# Autodesk Inventor assembly: use this - gimme that tech award
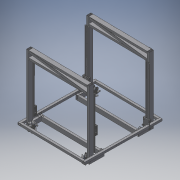
[picture p0: Inventor's stored thumbnail of the model, 180x180]
Saved by Autodesk Inventor 2018 (Build 220112000, 112)
## iProperties
Created: 2019-01-10
Part Number: use this - gimme that tech award
Document SubType Name: Assembly
Designer: maste
Author: maste
## Documents named in this file (7)
- \\studenthome\students\S-2512711\GitHub\2019CAD\Drivebase but Calvin is a mad man\use this - gimme that tech award.iam
- \\studenthome\students\S-2512711\GitHub\2019CAD\Drivebase but Calvin is a mad man\Slidey Mecanum L thing V2.iam
- \\studenthome\students\S-2512711\GitHub\2019CAD\Drivebase but Calvin is a mad man\1x1 30in.ipt
- \\studenthome\students\S-2512711\GitHub\2019CAD\Drivebase but Calvin is a mad man\1x1 35in.ipt
- \\studenthome\students\S-2512711\GitHub\2019CAD\Drivebase but Calvin is a mad man\1x1 L brackets 2in.ipt
- \\studenthome\students\S-2512711\GitHub\2019CAD\Drivebase but Calvin is a mad man\98404A101_18-8 STAINLESS STEEL QUICK-RELEASE PIN.ipt
- \\studenthome\students\S-2512711\GitHub\2019CAD\Drivebase but Calvin is a mad man\WW_10_40_10_AL_2.ipt
## Components (18 placed, 6 different names)
1. Slidey Mecanum L thing V2:1 [sub-assembly] — Mate:29, Mate:30, Flush:20, Flush:22, Flush:24, Mate:54, Mate:59, Mate:60, Mate:61, Mate:62
2. Slidey Mecanum L thing V2:2 [sub-assembly] — Flush:21, Mate:42, Flush:23, Mate:53, Flush:29, Mate:55, Mate:56, Mate:57, Mate:58
3. 1x1 30in:1 — Mate:31, Mate:32, Mate:33, Mate:34, Mate:35, Mate:36
4. 1x1 30in:2 — Mate:37, Mate:38, Mate:39, Flush:29
5. 1x1 35in:1 — Mate:29, Mate:30, Flush:20, Mate:31, Mate:32, Mate:33, Mate:45, Mate:46, Mate:47, Mate:48, Mate:54
6. 1x1 35in:2 — Mate:34, Mate:35, Mate:36, Mate:37, Mate:38, Mate:39, Mate:40, Mate:41, Mate:42, Mate:43, Mate:44, Mate:53
7. 1x1 L brackets 2in:1 — Flush:22, Mate:43, Mate:44, Mate:50, Flush:27, Rotation:2
8. 1x1 L brackets 2in:2 — Mate:40, Mate:41, Flush:21, Mate:49, Flush:28, Rotation:1
9. 1x1 L brackets 2in:3 — Mate:45, Mate:46, Flush:23, Mate:52, Flush:25, Rotation:4
10. 1x1 L brackets 2in:4 — Mate:47, Mate:48, Flush:24, Mate:51, Flush:26, Rotation:3
11. 98404A101_18-8 STAINLESS STEEL QUICK-RELEASE PIN:1 — Mate:52, Flush:25, Rotation:4
12. 98404A101_18-8 STAINLESS STEEL QUICK-RELEASE PIN:2 — Mate:51, Flush:26, Rotation:3
13. 98404A101_18-8 STAINLESS STEEL QUICK-RELEASE PIN:3 — Mate:50, Flush:27, Rotation:2
14. 98404A101_18-8 STAINLESS STEEL QUICK-RELEASE PIN:4 — Mate:49, Flush:28, Rotation:1
15. WW_10_40_10_AL_2:1 — Mate:57, Mate:58
16. WW_10_40_10_AL_2:2 — Mate:59, Mate:60
17. WW_10_40_10_AL_2:3 — Mate:61, Mate:62
18. WW_10_40_10_AL_2:4 — Mate:55, Mate:56
## Relationships (48: Mate 34, Flush 10, RelateRotation 4)
- Mate:29: Slidey Mecanum L thing V2:1 ↔ 1x1 35in:1
- Mate:30: Slidey Mecanum L thing V2:1 ↔ 1x1 35in:1
- Flush:20 (-76.2 mm): Slidey Mecanum L thing V2:1 ↔ 1x1 35in:1
- Mate:31: 1x1 30in:1 ↔ 1x1 35in:1
- Mate:32: 1x1 30in:1 ↔ 1x1 35in:1
- Mate:33: 1x1 30in:1 ↔ 1x1 35in:1
- Mate:34: 1x1 30in:1 ↔ 1x1 35in:2
- Mate:35: 1x1 30in:1 ↔ 1x1 35in:2
- Mate:36: 1x1 30in:1 ↔ 1x1 35in:2
- Mate:37: 1x1 30in:2 ↔ 1x1 35in:2
- Mate:38: 1x1 30in:2 ↔ 1x1 35in:2
- Mate:39: 1x1 30in:2 ↔ 1x1 35in:2
- Mate:40: 1x1 35in:2 ↔ 1x1 L brackets 2in:2
- Mate:41: 1x1 35in:2 ↔ 1x1 L brackets 2in:2
- Flush:21: Slidey Mecanum L thing V2:2 ↔ 1x1 L brackets 2in:2
- Mate:42: Slidey Mecanum L thing V2:2 ↔ 1x1 35in:2
- Flush:22: Slidey Mecanum L thing V2:1 ↔ 1x1 L brackets 2in:1
- Mate:43: 1x1 35in:2 ↔ 1x1 L brackets 2in:1
- Mate:44: 1x1 35in:2 ↔ 1x1 L brackets 2in:1
- Mate:45: 1x1 35in:1 ↔ 1x1 L brackets 2in:3
- Mate:46: 1x1 35in:1 ↔ 1x1 L brackets 2in:3
- Flush:23: Slidey Mecanum L thing V2:2 ↔ 1x1 L brackets 2in:3
- Mate:47: 1x1 35in:1 ↔ 1x1 L brackets 2in:4
- Mate:48: 1x1 35in:1 ↔ 1x1 L brackets 2in:4
- Flush:24: Slidey Mecanum L thing V2:1 ↔ 1x1 L brackets 2in:4
- Mate:49: 1x1 L brackets 2in:2 ↔ 98404A101_18-8 STAINLESS STEEL QUICK-RELEASE PIN:4
- Mate:50: 1x1 L brackets 2in:1 ↔ 98404A101_18-8 STAINLESS STEEL QUICK-RELEASE PIN:3
- Mate:51: 1x1 L brackets 2in:4 ↔ 98404A101_18-8 STAINLESS STEEL QUICK-RELEASE PIN:2
- Mate:52: 1x1 L brackets 2in:3 ↔ 98404A101_18-8 STAINLESS STEEL QUICK-RELEASE PIN:1
- Flush:25 (-10.16 mm): 1x1 L brackets 2in:3 ↔ 98404A101_18-8 STAINLESS STEEL QUICK-RELEASE PIN:1
- Flush:26 (-10.16 mm): 1x1 L brackets 2in:4 ↔ 98404A101_18-8 STAINLESS STEEL QUICK-RELEASE PIN:2
- Flush:27 (-10.16 mm): 1x1 L brackets 2in:1 ↔ 98404A101_18-8 STAINLESS STEEL QUICK-RELEASE PIN:3
- Flush:28 (-10.16 mm): 1x1 L brackets 2in:2 ↔ 98404A101_18-8 STAINLESS STEEL QUICK-RELEASE PIN:4
- Rotation:1 [RelateRotation] (1 ul): 1x1 L brackets 2in:2 ↔ 98404A101_18-8 STAINLESS STEEL QUICK-RELEASE PIN:4
- Rotation:2 [RelateRotation] (1 ul): 1x1 L brackets 2in:1 ↔ 98404A101_18-8 STAINLESS STEEL QUICK-RELEASE PIN:3
- Rotation:3 [RelateRotation] (1 ul): 1x1 L brackets 2in:4 ↔ 98404A101_18-8 STAINLESS STEEL QUICK-RELEASE PIN:2
- Rotation:4 [RelateRotation] (1 ul): 1x1 L brackets 2in:3 ↔ 98404A101_18-8 STAINLESS STEEL QUICK-RELEASE PIN:1
- Mate:53: Slidey Mecanum L thing V2:2 ↔ 1x1 35in:2
- Mate:54: Slidey Mecanum L thing V2:1 ↔ 1x1 35in:1
- Flush:29 (-76.2 mm): Slidey Mecanum L thing V2:2 ↔ 1x1 30in:2
- Mate:55: Slidey Mecanum L thing V2:2 ↔ WW_10_40_10_AL_2:4
- Mate:56: Slidey Mecanum L thing V2:2 ↔ WW_10_40_10_AL_2:4
- Mate:57: Slidey Mecanum L thing V2:2 ↔ WW_10_40_10_AL_2:1
- Mate:58: Slidey Mecanum L thing V2:2 ↔ WW_10_40_10_AL_2:1
- Mate:59: Slidey Mecanum L thing V2:1 ↔ WW_10_40_10_AL_2:2
- Mate:60: Slidey Mecanum L thing V2:1 ↔ WW_10_40_10_AL_2:2
- Mate:61: Slidey Mecanum L thing V2:1 ↔ WW_10_40_10_AL_2:3
- Mate:62: Slidey Mecanum L thing V2:1 ↔ WW_10_40_10_AL_2:3
